# Autodesk Inventor assembly: goalStructure
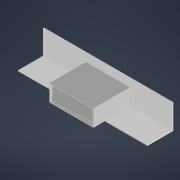
[picture p0: Inventor's stored thumbnail of the model, 180x180]
Saved by Autodesk Inventor 2021.4 (Build 254397000, 397)
## iProperties
Created: 2022-03-22
Part Number: goalStructure
Document SubType Name: Assembly
Designer: jo_ki
Author: jo_ki
## Documents named in this file (8)
- D:\Repos\SmartSoccerTableCAD\Parts\goalStructure\goalStructure.iam
- D:\Repos\SmartSoccerTableCAD\Parts\goalStructure\goalPanelFront.ipt
- D:\Repos\SmartSoccerTableCAD\Parts\goalStructure\goalPanelTop.ipt
- D:\Repos\SmartSoccerTableCAD\Parts\goalStructure\TorraumFrontKlein.ipt
- D:\Repos\SmartSoccerTableCAD\Parts\goalStructure\TorraumHinten.ipt
- D:\Repos\SmartSoccerTableCAD\Parts\goalStructure\TorraumSchrägeOben.ipt
- D:\Repos\SmartSoccerTableCAD\Parts\goalStructure\TorraumSeitenplatte.ipt
- D:\Repos\SmartSoccerTableCAD\Parts\goalStructure\goalPanelBottomSlope.ipt
## Components (8 placed, 7 different names)
1. goalPanelFront:1 — Flush:1, Mate:1, Flush:2, Mate:3, Flush:3, Mate:5, Mate:6, Flush:4, Mate:7, Mate:8, Mate:13
2. goalPanelTop:1 — Flush:1, Mate:1, Flush:2, Mate:2, Mate:4, Mate:11
3. TorraumFrontKlein:1 — Mate:12, Mate:13, Flush:6
4. TorraumHinten:1 — Mate:10, Mate:11, Flush:5, Mate:14
5. TorraumSchrägeOben:1 — Mate:7, Mate:8, Mate:9
6. TorraumSeitenplatte:1 — Mate:2, Mate:3, Flush:3, Mate:10, Flush:5, Mate:12, Flush:6
7. TorraumSeitenplatte:2 — Mate:4, Mate:5, Mate:6, Flush:4, Mate:9, Mate:15
8. goalPanelBottomSlope:1 — Mate:14, Mate:15
## Relationships (21: Mate 15, Flush 6)
- Flush:1: goalPanelFront:1 ↔ goalPanelTop:1
- Mate:1: goalPanelFront:1 ↔ goalPanelTop:1
- Flush:2: goalPanelFront:1 ↔ goalPanelTop:1
- Mate:2: goalPanelTop:1 ↔ TorraumSeitenplatte:1
- Mate:3: goalPanelFront:1 ↔ TorraumSeitenplatte:1
- Flush:3: goalPanelFront:1 ↔ TorraumSeitenplatte:1
- Mate:4: goalPanelTop:1 ↔ TorraumSeitenplatte:2
- Mate:5: goalPanelFront:1 ↔ TorraumSeitenplatte:2
- Mate:6: goalPanelFront:1 ↔ TorraumSeitenplatte:2
- Flush:4: goalPanelFront:1 ↔ TorraumSeitenplatte:2
- Mate:7: goalPanelFront:1 ↔ TorraumSchrägeOben:1
- Mate:8: goalPanelFront:1 ↔ TorraumSchrägeOben:1
- Mate:9: TorraumSchrägeOben:1 ↔ TorraumSeitenplatte:2
- Mate:10: TorraumHinten:1 ↔ TorraumSeitenplatte:1
- Mate:11: goalPanelTop:1 ↔ TorraumHinten:1
- Flush:5: TorraumHinten:1 ↔ TorraumSeitenplatte:1
- Mate:12: TorraumFrontKlein:1 ↔ TorraumSeitenplatte:1
- Mate:13: goalPanelFront:1 ↔ TorraumFrontKlein:1
- Flush:6: TorraumFrontKlein:1 ↔ TorraumSeitenplatte:1
- Mate:14: TorraumHinten:1 ↔ goalPanelBottomSlope:1
- Mate:15: TorraumSeitenplatte:2 ↔ goalPanelBottomSlope:1
